# Autodesk Inventor assembly: Robotic Gripper
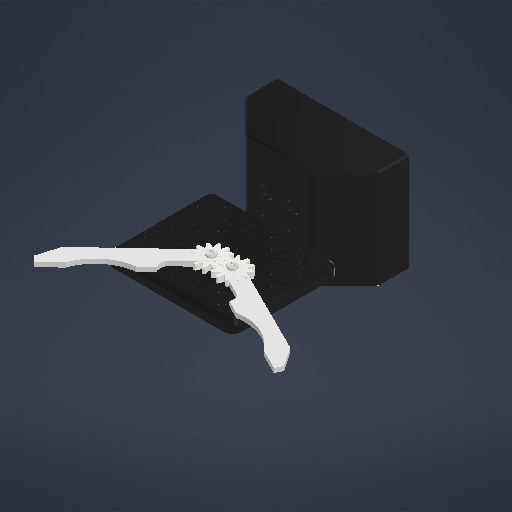
[picture p0: Inventor's stored thumbnail of the model, 512x512]
Saved by Autodesk Inventor 2026.1 (Build 301233000, 233)
## iProperties
Created: 2025-11-19
Part Number: Robotic Gripper
Document SubType Name: Assembly
Designer: auric
Author: auric
## Documents named in this file (6)
- C:\Users\auric\Downloads\Robotic Gripper.iam
- C:\Users\auric\Downloads\End Effector Platform Body.ipt
- C:\Users\auric\Downloads\robotic claw.ipt
- C:\Users\auric\Downloads\End Effector Platform\Fasteners\Steel M3x16 Pan Head Screw.ipt
- C:\Users\auric\Downloads\Robotic Gripper\Design Accelerator\Spur Gears1.iam
- C:\Users\auric\Downloads\End Effector Platform\Fasteners\Steel M3 Hex Nut.ipt
## Components (9 placed, 5 different names)
1. robotic claw:1 — Mate:1, Rotation:1, Flush:1, Insert:1
2. End Effector Platform Body:1 — Angle:1, Rotational:1, Rotational:2, Insert:3, Insert:4
3. Steel M3x16 Pan Head Screw:1 — Insert:1
4. Spur Gears:1 [sub-assembly] — Angle:1, Rotational:1, Mate:1, Rotation:1, Flush:1, Rotation:3
5. Steel M3x16 Pan Head Screw:2 — Insert:2
6. Spur Gears:2 [sub-assembly] — Rotational:2, Mate:2, Flush:2, Rotation:2, Rotation:3, Insert:2
7. robotic claw:2 — Mate:2, Flush:2, Rotation:2
8. Steel M3 Hex Nut:1 — Insert:3
9. Steel M3 Hex Nut:2 — Insert:4
## Relationships (14: Insert 4, RelateRotation 3, RevoluteJoint 2, Mate 2, Flush 2, Angle 1)
- Angle:1 (0 deg): End Effector Platform Body:1 ↔ Spur Gears:1
- Rotational:1 [RevoluteJoint]: End Effector Platform Body:1 ↔ Spur Gears:1
- Mate:1: robotic claw:1 ↔ Spur Gears:1
- Rotation:1 [RelateRotation] (1 ul): robotic claw:1 ↔ Spur Gears:1
- Flush:1: robotic claw:1 ↔ Spur Gears:1
- Insert:1: robotic claw:1 ↔ Steel M3x16 Pan Head Screw:1
- Rotational:2 [RevoluteJoint]: End Effector Platform Body:1 ↔ Spur Gears:2
- Mate:2: Spur Gears:2 ↔ robotic claw:2
- Flush:2: Spur Gears:2 ↔ robotic claw:2
- Rotation:2 [RelateRotation] (1 ul): Spur Gears:2 ↔ robotic claw:2
- Rotation:3 [RelateRotation] (1 ul): Spur Gears:1 ↔ Spur Gears:2
- Insert:2: Steel M3x16 Pan Head Screw:2 ↔ Spur Gears:2
- Insert:3: End Effector Platform Body:1 ↔ Steel M3 Hex Nut:1
- Insert:4: End Effector Platform Body:1 ↔ Steel M3 Hex Nut:2
